# Autodesk Inventor assembly: weldments1
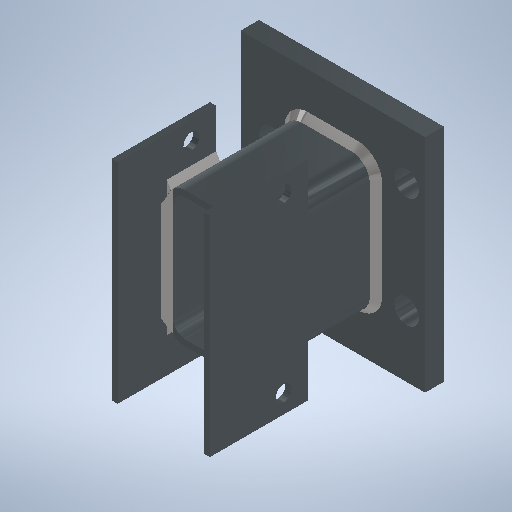
[picture p0: Inventor's stored thumbnail of the model, 512x512]
Saved by Autodesk Inventor 2025.2 (Build 292293000, 293)
## iProperties
Created: 2025-03-25
Part Number: weldments1
Document SubType Name: Weldment
Designer: bless
Weld Material: Steel, Mild
Author: bless
## Documents named in this file (5)
- C:\Users\bless\OneDrive - Conestoga College\Documents\Inventor\8071W25\weldmants\weldments1.iam
- C:\Users\bless\OneDrive - Conestoga College\Documents\Inventor\8071W25\weldmants\class1 (1).ipt
- C:\Users\bless\OneDrive - Conestoga College\Documents\Inventor\8071W25\weldmants\class2 (1).ipt
- C:\Users\bless\OneDrive - Conestoga College\Documents\Inventor\8071W25\weldmants\class3 (1).ipt
- C:\Users\bless\OneDrive - Conestoga College\Documents\Inventor\8071W25\weldmants\class3 (1)_MIR1.ipt
## Components (4 placed, 4 different names)
1. class1 (1):1 — Mate:1, Flush:1, Flush:2, Mate:2, Flush:3
2. class2 (1):1 — Mate:1, Flush:1, Flush:2
3. class3 (1):1 — Mate:2, Flush:3
4. class3 (1)_MIR1:1
## Relationships (5: Flush 3, Mate 2)
- Mate:1: class1 (1):1 ↔ class2 (1):1
- Flush:1 (44.45 mm): class1 (1):1 ↔ class2 (1):1
- Flush:2 (50.8 mm): class1 (1):1 ↔ class2 (1):1
- Mate:2: class1 (1):1 ↔ class3 (1):1
- Flush:3 (50.8 mm): class1 (1):1 ↔ class3 (1):1
